# Autodesk Inventor assembly: 基本構造
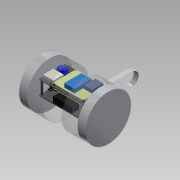
[picture p0: Inventor's stored thumbnail of the model, 180x180]
Saved by Autodesk Inventor 2017 (Build 210142000, 142)
## iProperties
Part Number: 基本構造
Material: 一般
Document SubType Name: Assembly
Designer: HISAAKI
Author: HISAAKI
## Documents named in this file (19)
- C:\Users\HISAAKI\Documents\LYNCS\CanSat\2017種子島\cansat-structure\基本構造.iam
- C:\Users\HISAAKI\Documents\LYNCS\CanSat\2017種子島\cansat-structure\基本板.ipt
- C:\Users\HISAAKI\Documents\LYNCS\CanSat\2017種子島\cansat-structure\既成部品\ブラケット.ipt
- C:\Users\HISAAKI\Documents\LYNCS\CanSat\2017種子島\cansat-structure\既成部品\モータ.ipt
- C:\Users\HISAAKI\Documents\LYNCS\CanSat\2017種子島\cansat-structure\ハブver1.1.ipt
- C:\Users\HISAAKI\Documents\LYNCS\CanSat\2017種子島\cansat-structure\タイヤスポンジ部分.ipt
- C:\Users\HISAAKI\Documents\LYNCS\CanSat\2017種子島\cansat-structure\既成部品\リポ電池.ipt
- C:\Users\HISAAKI\Documents\LYNCS\CanSat\2017種子島\cansat-structure\基本板上.ipt
- C:\Users\HISAAKI\Documents\LYNCS\CanSat\2017種子島\cansat-structure\既成部品\mbed.ipt
- C:\Users\HISAAKI\Documents\LYNCS\CanSat\2017種子島\cansat-structure\既成部品\スペーサ.ipt
- C:\Users\HISAAKI\Documents\LYNCS\CanSat\2017種子島\cansat-structure\既成部品\GPSユニット.ipt
- C:\Users\HISAAKI\Documents\LYNCS\CanSat\2017種子島\cansat-structure\距離センサ.ipt
- C:\Users\HISAAKI\Documents\LYNCS\CanSat\2017種子島\cansat-structure\xBee.ipt
- C:\Users\HISAAKI\Documents\LYNCS\CanSat\2017種子島\cansat-structure\基板.ipt
- C:\Users\HISAAKI\Documents\LYNCS\CanSat\2017種子島\cansat-structure\スペーサ5mm.ipt
- C:\Users\HISAAKI\Documents\LYNCS\CanSat\2017種子島\cansat-structure\タイヤプラ板部分.ipt
- C:\Users\HISAAKI\Documents\LYNCS\CanSat\2017種子島\cansat-structure\サーボ.ipt
- C:\Users\HISAAKI\Documents\LYNCS\CanSat\2017種子島\cansat-structure\スタビライザ.ipt
- C:\Users\HISAAKI\Documents\LYNCS\CanSat\2017種子島\cansat-structure\モータドライバ.ipt
## Components (35 placed, 18 different names)
1. 基本板:1 — フラッシュ:1, フラッシュ:2, メイト:19, メイト:20, メイト:21, メイト:23, メイト:24, メイト:25, メイト:26, メイト:27, メイト:28, メイト:29, メイト:30, フラッシュ:4, フラッシュ:6, メイト:35, メイト:36, メイト:37, メイト:38, メイト:39, メイト:40, フラッシュ:7, メイト:46, メイト:77, メイト:85, メイト:86, メイト:87
2. モータ:1 — フラッシュ:2, メイト:13, メイト:14, メイト:41, メイト:43
3. モータ:2 — フラッシュ:1, メイト:11, メイト:12, メイト:42, メイト:44
4. ハブver1.1:1 — メイト:11, メイト:12, メイト:17, メイト:18
5. ハブver1.1:2 — メイト:13, メイト:14, メイト:15, メイト:16
6. タイヤスポンジ部分:1 — メイト:15, メイト:16, メイト:62, メイト:63
7. タイヤスポンジ部分:2 — メイト:17, メイト:18, メイト:64, メイト:65
8. リポ電池:1 — メイト:19, フラッシュ:4, フラッシュ:6
9. 基本板上:1 — メイト:20, メイト:21, メイト:31, メイト:32, フラッシュ:5, メイト:47, メイト:48, メイト:49, メイト:50, メイト:51, メイト:52, メイト:53, メイト:54, メイト:66, メイト:67, メイト:68, メイト:69, メイト:70, メイト:71, メイト:72, メイト:73, メイト:79, メイト:80, メイト:81
10. スペーサ:1 — メイト:23, メイト:29
11. スペーサ:2 — メイト:25, メイト:28
12. スペーサ:3 — メイト:24, メイト:30, メイト:31
13. スペーサ:4 — メイト:26, メイト:27
14. GPSユニット:1 — メイト:32, フラッシュ:5
15. ブラケット:1 — メイト:35, メイト:36, メイト:37, メイト:41, メイト:43
16. ブラケット:2 — メイト:38, メイト:39, メイト:40, メイト:42, メイト:44
17. 距離センサ:1 — フラッシュ:7, メイト:46
18. スペーサ5mm:1 — メイト:47, メイト:51, メイト:58
19. スペーサ5mm:2 — メイト:50, メイト:52, メイト:57
20. スペーサ5mm:3 — メイト:48, メイト:54, メイト:55, メイト:59
21. スペーサ5mm:4 — メイト:49, メイト:53, メイト:56
22. 基板:1 — メイト:55, メイト:56, メイト:57, メイト:58, メイト:59, メイト:60, メイト:61, フラッシュ:9, フラッシュ:10, フラッシュ:11
23. mbed:1 — メイト:60, フラッシュ:11
24. xBee:1 — メイト:61, フラッシュ:9, フラッシュ:10
25. タイヤプラ板部分:1 — メイト:62, メイト:63
26. タイヤプラ板部分:2 — メイト:64, メイト:65
27. スペーサ5mm:5 — メイト:66, メイト:72
28. スペーサ5mm:6 — メイト:68, メイト:73, メイト:74
29. スペーサ5mm:7 — メイト:67, メイト:70, メイト:75, メイト:76
30. スペーサ5mm:8 — メイト:69, メイト:71
31. 基板:2 — メイト:74, メイト:75, メイト:76, メイト:82, フラッシュ:13, メイト:84
32. スタビライザ:1 — メイト:77, メイト:85, メイト:86, メイト:87
33. サーボ:1 — メイト:79, メイト:80, メイト:81
34. モータドライバ:1 — フラッシュ:12, メイト:83, フラッシュ:14, メイト:84
35. モータドライバ:2 — フラッシュ:12, メイト:82, フラッシュ:13, メイト:83, フラッシュ:14
## Relationships (84: Mate 72, Flush 12)
- フラッシュ:1 [Flush]: 基本板:1 ↔ モータ:2
- フラッシュ:2 [Flush]: 基本板:1 ↔ モータ:1
- メイト:11 [Mate]: モータ:2 ↔ ハブver1.1:1
- メイト:12 [Mate]: モータ:2 ↔ ハブver1.1:1
- メイト:13 [Mate]: モータ:1 ↔ ハブver1.1:2
- メイト:14 [Mate]: モータ:1 ↔ ハブver1.1:2
- メイト:15 [Mate]: ハブver1.1:2 ↔ タイヤスポンジ部分:1
- メイト:16 [Mate]: ハブver1.1:2 ↔ タイヤスポンジ部分:1
- メイト:17 [Mate]: ハブver1.1:1 ↔ タイヤスポンジ部分:2
- メイト:18 [Mate]: ハブver1.1:1 ↔ タイヤスポンジ部分:2
- メイト:19 [Mate]: 基本板:1 ↔ リポ電池:1
- メイト:20 [Mate]: 基本板:1 ↔ 基本板上:1
- メイト:21 [Mate]: 基本板:1 ↔ 基本板上:1
- メイト:23 [Mate]: 基本板:1 ↔ スペーサ:1
- メイト:24 [Mate]: 基本板:1 ↔ スペーサ:3
- メイト:25 [Mate]: 基本板:1 ↔ スペーサ:2
- メイト:26 [Mate]: 基本板:1 ↔ スペーサ:4
- メイト:27 [Mate]: 基本板:1 ↔ スペーサ:4
- メイト:28 [Mate]: 基本板:1 ↔ スペーサ:2
- メイト:29 [Mate]: 基本板:1 ↔ スペーサ:1
- メイト:30 [Mate]: 基本板:1 ↔ スペーサ:3
- メイト:31 [Mate]: 基本板上:1 ↔ スペーサ:3
- メイト:32 [Mate]: 基本板上:1 ↔ GPSユニット:1
- フラッシュ:4 [Flush] (40 mm): 基本板:1 ↔ リポ電池:1
- フラッシュ:5 [Flush] (10 mm): 基本板上:1 ↔ GPSユニット:1
- フラッシュ:6 [Flush] (36 mm): 基本板:1 ↔ リポ電池:1
- メイト:35 [Mate]: 基本板:1 ↔ ブラケット:1
- メイト:36 [Mate]: 基本板:1 ↔ ブラケット:1
- メイト:37 [Mate]: 基本板:1 ↔ ブラケット:1
- メイト:38 [Mate]: 基本板:1 ↔ ブラケット:2
- メイト:39 [Mate]: 基本板:1 ↔ ブラケット:2
- メイト:40 [Mate]: 基本板:1 ↔ ブラケット:2
- メイト:41 [Mate]: モータ:1 ↔ ブラケット:1
- メイト:42 [Mate]: モータ:2 ↔ ブラケット:2
- メイト:43 [Mate]: モータ:1 ↔ ブラケット:1
- メイト:44 [Mate]: モータ:2 ↔ ブラケット:2
- フラッシュ:7 [Flush]: 基本板:1 ↔ 距離センサ:1
- メイト:46 [Mate]: 基本板:1 ↔ 距離センサ:1
- メイト:47 [Mate]: 基本板上:1 ↔ スペーサ5mm:1
- メイト:48 [Mate]: 基本板上:1 ↔ スペーサ5mm:3
- メイト:49 [Mate]: 基本板上:1 ↔ スペーサ5mm:4
- メイト:50 [Mate]: 基本板上:1 ↔ スペーサ5mm:2
- メイト:51 [Mate]: 基本板上:1 ↔ スペーサ5mm:1
- メイト:52 [Mate]: 基本板上:1 ↔ スペーサ5mm:2
- メイト:53 [Mate]: 基本板上:1 ↔ スペーサ5mm:4
- メイト:54 [Mate]: 基本板上:1 ↔ スペーサ5mm:3
- メイト:55 [Mate]: スペーサ5mm:3 ↔ 基板:1
- メイト:56 [Mate]: スペーサ5mm:4 ↔ 基板:1
- メイト:57 [Mate]: スペーサ5mm:2 ↔ 基板:1
- メイト:58 [Mate]: スペーサ5mm:1 ↔ 基板:1
- メイト:59 [Mate]: スペーサ5mm:3 ↔ 基板:1
- メイト:60 [Mate]: 基板:1 ↔ mbed:1
- メイト:61 [Mate]: 基板:1 ↔ xBee:1
- フラッシュ:9 [Flush] (5 mm): 基板:1 ↔ xBee:1
- フラッシュ:10 [Flush] (5 mm): 基板:1 ↔ xBee:1
- フラッシュ:11 [Flush] (5 mm): 基板:1 ↔ mbed:1
- メイト:62 [Mate]: タイヤスポンジ部分:1 ↔ タイヤプラ板部分:1
- メイト:63 [Mate]: タイヤスポンジ部分:1 ↔ タイヤプラ板部分:1
- メイト:64 [Mate]: タイヤスポンジ部分:2 ↔ タイヤプラ板部分:2
- メイト:65 [Mate]: タイヤスポンジ部分:2 ↔ タイヤプラ板部分:2
- メイト:66 [Mate]: 基本板上:1 ↔ スペーサ5mm:5
- メイト:67 [Mate]: 基本板上:1 ↔ スペーサ5mm:7
- メイト:68 [Mate]: 基本板上:1 ↔ スペーサ5mm:6
- メイト:69 [Mate]: 基本板上:1 ↔ スペーサ5mm:8
- メイト:70 [Mate]: 基本板上:1 ↔ スペーサ5mm:7
- メイト:71 [Mate]: 基本板上:1 ↔ スペーサ5mm:8
- メイト:72 [Mate]: 基本板上:1 ↔ スペーサ5mm:5
- メイト:73 [Mate]: 基本板上:1 ↔ スペーサ5mm:6
- メイト:74 [Mate]: スペーサ5mm:6 ↔ 基板:2
- メイト:75 [Mate]: スペーサ5mm:7 ↔ 基板:2
- メイト:76 [Mate]: スペーサ5mm:7 ↔ 基板:2
- メイト:77 [Mate]: 基本板:1 ↔ スタビライザ:1
- メイト:79 [Mate]: 基本板上:1 ↔ サーボ:1
- メイト:80 [Mate]: 基本板上:1 ↔ サーボ:1
- メイト:81 [Mate]: 基本板上:1 ↔ サーボ:1
- フラッシュ:12 [Flush]: モータドライバ:1 ↔ モータドライバ:2
- メイト:82 [Mate]: 基板:2 ↔ モータドライバ:2
- フラッシュ:13 [Flush] (5 mm): 基板:2 ↔ モータドライバ:2
- メイト:83 [Mate] (5 mm): モータドライバ:1 ↔ モータドライバ:2
- フラッシュ:14 [Flush]: モータドライバ:1 ↔ モータドライバ:2
- メイト:84 [Mate] (5 mm): 基板:2 ↔ モータドライバ:1
- メイト:85 [Mate] (-30 mm): 基本板:1 ↔ スタビライザ:1
- メイト:86 [Mate]: 基本板:1 ↔ スタビライザ:1
- メイト:87 [Mate]: 基本板:1 ↔ スタビライザ:1
